# Autodesk Inventor assembly: Funnel Plate Assembly
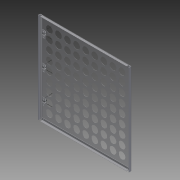
[picture p0: Inventor's stored thumbnail of the model, 180x180]
Saved by Autodesk Inventor 2014 (Build 180170000, 170)
## iProperties
Created: 2014-01-05
Part Number: Funnel Plate Assembly
Document SubType Name: Assembly
Designer: Michael
Author: Michael
## Documents named in this file (6)
- C:\Users\Michael\Documents\Robotics\2014 Season\Prep CAD\Funnel Plate Assembly.iam
- C:\Users\Michael\Documents\Robotics\2014 Season\Prep CAD\Plastic Funnel PIece.ipt
- C:\Users\Michael\Documents\Robotics\2014 Season\Prep CAD\.05 in Aluminum Angle.ipt
- C:\Users\Michael\Documents\Robotics\2014 Season\Prep CAD\.05 in Aluminum Angle (19 in).ipt
- C:\Users\Michael\Documents\Robotics\2014 Season\Prep CAD\Flange for Torsion Spring.ipt
- C:\Users\Michael\Documents\Robotics\2014 Season\Prep CAD\Torsion Spring  (9271K586).ipt
## Components (14 placed, 5 different names)
1. Plastic Funnel PIece:1 — Insert:9, Insert:10, Insert:13, Insert:14, Insert:15, Insert:16, Insert:17, Insert:18, Insert:19, Insert:20, Insert:21, Insert:22, Angle:1, Insert:23, Insert:24, Insert:25, Insert:26, Insert:27, Insert:28, Insert:29, Insert:30
2. .05 in Aluminum Angle:1 — Insert:25, Insert:26
3. .05 in Aluminum Angle:2 — Insert:23, Insert:24
4. .05 in Aluminum Angle (19 in):1 — Insert:27, Insert:28
5. .05 in Aluminum Angle (19 in):2 — Insert:29, Insert:30
6. Flange for Torsion Spring:1 — Insert:19, Insert:20, Mate:6
7. Flange for Torsion Spring:2 — Insert:17, Insert:18, Mate:2, Angle:2
8. Flange for Torsion Spring:3 — Insert:21, Insert:22, Mate:1
9. Flange for Torsion Spring:4 — Insert:15, Insert:16, Angle:3
10. Flange for Torsion Spring:5 — Insert:13, Insert:14, Mate:5
11. Flange for Torsion Spring:7 — Insert:9, Insert:10, Mate:3, Mate:4
12. Torsion Spring  (9271K586):1 — Mate:1, Angle:1, Mate:6
13. Torsion Spring  (9271K586):2 — Mate:2, Angle:2, Mate:5
14. Torsion Spring  (9271K586):3 — Mate:3, Angle:3, Mate:4
## Relationships (29: Insert 20, Mate 6, Angle 3)
- Insert:9: Plastic Funnel PIece:1 ↔ Flange for Torsion Spring:7
- Insert:10: Plastic Funnel PIece:1 ↔ Flange for Torsion Spring:7
- Insert:13: Plastic Funnel PIece:1 ↔ Flange for Torsion Spring:5
- Insert:14: Plastic Funnel PIece:1 ↔ Flange for Torsion Spring:5
- Insert:15: Plastic Funnel PIece:1 ↔ Flange for Torsion Spring:4
- Insert:16: Plastic Funnel PIece:1 ↔ Flange for Torsion Spring:4
- Insert:17: Plastic Funnel PIece:1 ↔ Flange for Torsion Spring:2
- Insert:18: Plastic Funnel PIece:1 ↔ Flange for Torsion Spring:2
- Insert:19: Plastic Funnel PIece:1 ↔ Flange for Torsion Spring:1
- Insert:20: Plastic Funnel PIece:1 ↔ Flange for Torsion Spring:1
- Insert:21: Plastic Funnel PIece:1 ↔ Flange for Torsion Spring:3
- Insert:22: Plastic Funnel PIece:1 ↔ Flange for Torsion Spring:3
- Mate:1: Flange for Torsion Spring:3 ↔ Torsion Spring  (9271K586):1
- Angle:1 (0 deg): Plastic Funnel PIece:1 ↔ Torsion Spring  (9271K586):1
- Mate:2: Flange for Torsion Spring:2 ↔ Torsion Spring  (9271K586):2
- Angle:2 (0 deg): Flange for Torsion Spring:2 ↔ Torsion Spring  (9271K586):2
- Mate:3: Flange for Torsion Spring:7 ↔ Torsion Spring  (9271K586):3
- Angle:3 (0 deg): Flange for Torsion Spring:4 ↔ Torsion Spring  (9271K586):3
- Mate:4 (1.5875 mm): Flange for Torsion Spring:7 ↔ Torsion Spring  (9271K586):3
- Mate:5 (1.5875 mm): Flange for Torsion Spring:5 ↔ Torsion Spring  (9271K586):2
- Mate:6 (1.5875 mm): Flange for Torsion Spring:1 ↔ Torsion Spring  (9271K586):1
- Insert:23: Plastic Funnel PIece:1 ↔ .05 in Aluminum Angle:2
- Insert:24: Plastic Funnel PIece:1 ↔ .05 in Aluminum Angle:2
- Insert:25: Plastic Funnel PIece:1 ↔ .05 in Aluminum Angle:1
- Insert:26: Plastic Funnel PIece:1 ↔ .05 in Aluminum Angle:1
- Insert:27: Plastic Funnel PIece:1 ↔ .05 in Aluminum Angle (19 in):1
- Insert:28: Plastic Funnel PIece:1 ↔ .05 in Aluminum Angle (19 in):1
- Insert:29: Plastic Funnel PIece:1 ↔ .05 in Aluminum Angle (19 in):2
- Insert:30: Plastic Funnel PIece:1 ↔ .05 in Aluminum Angle (19 in):2
